# Autodesk Inventor assembly: Assemlby_OT2-Gripper
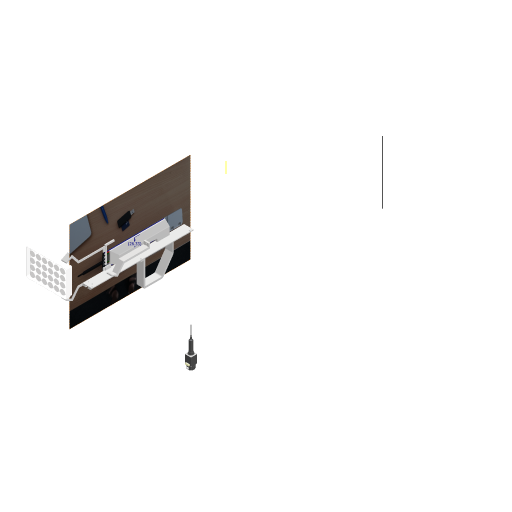
[picture p0: Inventor's stored thumbnail of the model, 512x512]
Saved by Autodesk Inventor 2024.1 (Build 281209000, 209)
## iProperties
Created: 2024-09-04
Part Number: Assemlby_OT2-Gripper
Document SubType Name: Assembly
Designer: diederichbenedict
Author: diederichbenedict
## Documents named in this file (11)
- C:\Users\diederichbenedict\Dropbox\Dokumente\Promotion\PROJECTS\openUC2-CAD\INVENTOR\Assemlby_OT2-Gripper.iam
- C:\Users\diederichbenedict\Dropbox\Dokumente\Promotion\PROJECTS\openUC2-CAD\INVENTOR\00_OT-2 Reference_Pipettte.ipt
- C:\Users\diederichbenedict\Dropbox\Dokumente\Promotion\PROJECTS\openUC2-CAD\INVENTOR\00_OT2-Pippette_1.ipt
- C:\Users\diederichbenedict\Dropbox\Dokumente\Promotion\PROJECTS\openUC2-CAD\INVENTOR\00_Joy-IT-B20SHD4353_NEMA8_captive.ipt
- C:\Users\diederichbenedict\Dropbox\Dokumente\Promotion\PROJECTS\openUC2-CAD\INVENTOR\00_24wellplate_base_2.ipt
- C:\Users\diederichbenedict\Dropbox\Dokumente\Promotion\PROJECTS\openUC2-CAD\INVENTOR\OT2-Gripper_base.ipt
- C:\Users\diederichbenedict\Dropbox\Dokumente\Promotion\PROJECTS\openUC2-CAD\INVENTOR\Actuator_MGN9.ipt
- C:\Users\diederichbenedict\Dropbox\Dokumente\Promotion\PROJECTS\openUC2-CAD\INVENTOR\Actuator_MGN9C.ipt
- C:\Users\diederichbenedict\Dropbox\Dokumente\Promotion\PROJECTS\openUC2-CAD\INVENTOR\OT2-Gripper_slider.ipt
- C:\Users\diederichbenedict\Dropbox\Dokumente\Promotion\PROJECTS\openUC2-CAD\INVENTOR\OT2-Gripper_block.ipt
- C:\Users\diederichbenedict\Dropbox\Dokumente\Promotion\PROJECTS\openUC2-CAD\INVENTOR\OT2-Gripper_finger.ipt
## Components (13 placed, 10 different names)
1. 00_OT-2 Reference_Pipettte:1 — Fluchtend:4, Passend:1, Passend:2, Passend:3, Passend:4, Fluchtend:5, Fluchtend:6, Fluchtend:7, Passend:5
2. 00_OT2-Pippette_1:1 — Fluchtend:4
3. 00_Joy-IT-B20SHD4353_NEMA8_captive:1 — Passend:3, Passend:4, Fluchtend:5, Fluchtend:8
4. 00_24wellplate_base_2:1 — Passend:1, Passend:2
5. 00_Joy-IT-B20SHD4353_NEMA8_captive:2
6. OT2-Gripper_base:1 — Fluchtend:6, Fluchtend:7, Fluchtend:8, Passend:6, Fluchtend:9
7. Actuator_MGN9:1 — Passend:5, Passend:6, Fluchtend:9, Fluchtend:10, Passend:7, Fluchtend:17
8. Actuator_MGN9C:1 — Fluchtend:10, Passend:7, Fluchtend:12, Fluchtend:13
9. OT2-Gripper_slider:1 — Fluchtend:12, Fluchtend:13, Einfügen:1, Winkel:1
10. OT2-Gripper_block:1 — Fluchtend:15, Fluchtend:16, Fluchtend:17
11. OT2-Gripper_finger:1 — Fluchtend:15, Fluchtend:16
12. OT2-Gripper_finger:2
13. OT2-Gripper_finger:3 — Einfügen:1, Winkel:1
## Relationships (21: Flush 12, Mate 7, Insert 1, Angle 1)
- Fluchtend:4 [Flush] (-17 mm): 00_OT-2 Reference_Pipettte:1 ↔ 00_OT2-Pippette_1:1
- Passend:1 [Mate]: 00_OT-2 Reference_Pipettte:1 ↔ 00_24wellplate_base_2:1
- Passend:2 [Mate] (125 mm): 00_OT-2 Reference_Pipettte:1 ↔ 00_24wellplate_base_2:1
- Passend:3 [Mate]: 00_OT-2 Reference_Pipettte:1 ↔ 00_Joy-IT-B20SHD4353_NEMA8_captive:1
- Passend:4 [Mate] (10 mm): 00_OT-2 Reference_Pipettte:1 ↔ 00_Joy-IT-B20SHD4353_NEMA8_captive:1
- Fluchtend:5 [Flush]: 00_OT-2 Reference_Pipettte:1 ↔ 00_Joy-IT-B20SHD4353_NEMA8_captive:1
- Fluchtend:6 [Flush]: 00_OT-2 Reference_Pipettte:1 ↔ OT2-Gripper_base:1
- Fluchtend:7 [Flush]: 00_OT-2 Reference_Pipettte:1 ↔ OT2-Gripper_base:1
- Fluchtend:8 [Flush]: 00_Joy-IT-B20SHD4353_NEMA8_captive:1 ↔ OT2-Gripper_base:1
- Passend:5 [Mate] (0.5 mm): 00_OT-2 Reference_Pipettte:1 ↔ Actuator_MGN9:1
- Passend:6 [Mate]: OT2-Gripper_base:1 ↔ Actuator_MGN9:1
- Fluchtend:9 [Flush]: OT2-Gripper_base:1 ↔ Actuator_MGN9:1
- Fluchtend:10 [Flush]: Actuator_MGN9:1 ↔ Actuator_MGN9C:1
- Passend:7 [Mate]: Actuator_MGN9:1 ↔ Actuator_MGN9C:1
- Fluchtend:12 [Flush]: Actuator_MGN9C:1 ↔ OT2-Gripper_slider:1
- Fluchtend:13 [Flush]: Actuator_MGN9C:1 ↔ OT2-Gripper_slider:1
- Fluchtend:15 [Flush]: OT2-Gripper_block:1 ↔ OT2-Gripper_finger:1
- Fluchtend:16 [Flush]: OT2-Gripper_block:1 ↔ OT2-Gripper_finger:1
- Einfügen:1 [Insert]: OT2-Gripper_slider:1 ↔ OT2-Gripper_finger:3
- Fluchtend:17 [Flush]: Actuator_MGN9:1 ↔ OT2-Gripper_block:1
- Winkel:1 [Angle] (0 deg): OT2-Gripper_slider:1 ↔ OT2-Gripper_finger:3
